# Autodesk Inventor assembly: Maquina
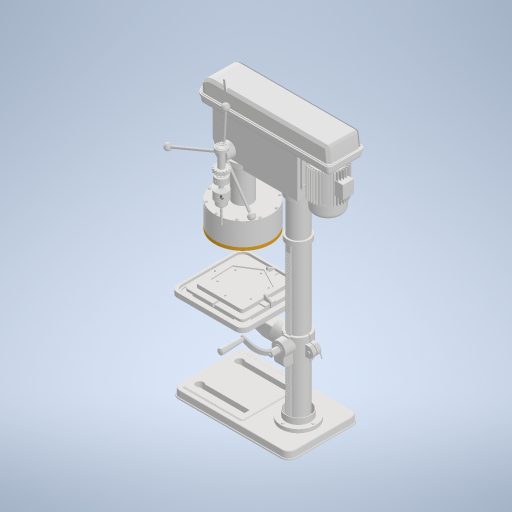
[picture p0: Inventor's stored thumbnail of the model, 512x512]
Saved by Autodesk Inventor 2024.2 (Build 282272000, 272)
## iProperties
Created: 2021-09-13
Part Number: Maquina
Description: STEP AP203
Document SubType Name: Assembly
Designer: 062210026
Sending System: SolidWorks 2018
Preprocessor: SwSTEP 2.0
Title: multi-spindle.STEP
Author: Moghimi
Revision Number: ANY
## Documents named in this file (37)
- C:\Users\062210029\Desktop\19MarV2_ProjInt3\19MarV2_ProjInt3\Maquina\Maquina.iam
- C:\Users\062210029\Desktop\19MarV2_ProjInt3\19MarV2_ProjInt3\Maquina\maquina\1_Varsay_lan.ipt
- C:\Users\062210029\Desktop\19MarV2_ProjInt3\19MarV2_ProjInt3\Maquina\maquina\2_Varsay_lan.ipt
- C:\Users\062210029\Desktop\19MarV2_ProjInt3\19MarV2_ProjInt3\Maquina\maquina\4_Varsay_lan.ipt
- C:\Users\062210029\Desktop\19MarV2_ProjInt3\19MarV2_ProjInt3\Maquina\maquina\5_Varsay_lan.ipt
- C:\Users\062210029\Desktop\19MarV2_ProjInt3\19MarV2_ProjInt3\Maquina\maquina\6_Varsay_lan.ipt
- C:\Users\062210029\Desktop\19MarV2_ProjInt3\19MarV2_ProjInt3\Maquina\maquina\7_Varsay_lan.ipt
- C:\Users\062210029\Desktop\19MarV2_ProjInt3\19MarV2_ProjInt3\Maquina\maquina\8_Varsay_lan.ipt
- C:\Users\062210029\Desktop\19MarV2_ProjInt3\19MarV2_ProjInt3\Maquina\maquina\9_Varsay_lan.ipt
- C:\Users\062210029\Desktop\19MarV2_ProjInt3\19MarV2_ProjInt3\Maquina\maquina\10_Varsay_lan.ipt
- C:\Users\062210029\Desktop\19MarV2_ProjInt3\19MarV2_ProjInt3\Maquina\maquina\11_Varsay_lan.ipt
- C:\Users\062210029\Desktop\19MarV2_ProjInt3\19MarV2_ProjInt3\Maquina\maquina\12_Varsay_lan.ipt
- C:\Users\062210029\Desktop\19MarV2_ProjInt3\19MarV2_ProjInt3\Maquina\maquina\13_Varsay_lan.ipt
- C:\Users\062210029\Desktop\19MarV2_ProjInt3\19MarV2_ProjInt3\Maquina\maquina\14_Varsay_lan.ipt
- C:\Users\062210029\Desktop\19MarV2_ProjInt3\19MarV2_ProjInt3\Maquina\maquina\15_Varsay_lan.ipt
- C:\Users\062210029\Desktop\19MarV2_ProjInt3\19MarV2_ProjInt3\Maquina\maquina\16_Varsay_lan.ipt
- C:\Users\062210029\Desktop\19MarV2_ProjInt3\19MarV2_ProjInt3\Maquina\maquina\hex bolt gradeab_iso_ISO 4014 - M4 x 35 x 14-N.ipt
- C:\Users\062210029\Desktop\19MarV2_ProjInt3\19MarV2_ProjInt3\Maquina\maquina\hex bolt gradeab_iso_ISO 4014 - M3 x 20 x 12-N.ipt
- C:\Users\062210029\Desktop\19MarV2_ProjInt3\19MarV2_ProjInt3\Maquina\maquina\hex bolt gradeab_iso_ISO 4014 - M6 x 30 x 18-N.ipt
- C:\Users\062210029\Desktop\19MarV2_ProjInt3\19MarV2_ProjInt3\Maquina\maquina\slotted cheese head screw_iso_ISO 1207 - M6 x 8 - 8N.ipt
- C:\Users\062210029\Desktop\19MarV2_ProjInt3\19MarV2_ProjInt3\Maquina\maquina\SKF_6004.iam
- C:\Users\062210029\Desktop\19MarV2_ProjInt3\19MarV2_ProjInt3\Maquina\maquina\MAILN AX.ipt
- C:\Users\062210029\Desktop\19MarV2_ProjInt3\19MarV2_ProjInt3\Maquina\maquina\SKF_30204.iam
- C:\Users\062210029\Desktop\19MarV2_ProjInt3\19MarV2_ProjInt3\Maquina\maquina\helical gear_3_am2_Metric - RH Helical gear 2.5M 30T 45HA 20PA 15FW ---30N75H50L35.0R1.ipt
- C:\Users\062210029\Desktop\19MarV2_ProjInt3\19MarV2_ProjInt3\Maquina\maquina\6-AX.ipt
- C:\Users\062210029\Desktop\19MarV2_ProjInt3\19MarV2_ProjInt3\Maquina\maquina\helical gear_3_am2_Metric - RH Helical gear 2.5M 15T 45HA 20PA 15FW ---15N75H50L25.0R1.ipt
- C:\Users\062210029\Desktop\19MarV2_ProjInt3\19MarV2_ProjInt3\Maquina\maquina\SHEL.ipt
- C:\Users\062210029\Desktop\19MarV2_ProjInt3\19MarV2_ProjInt3\Maquina\maquina\socket head cap screw_am_B18.3.1M - 5 x 0.8 x 20 Hex SHCS -- 20NHX.ipt
- C:\Users\062210029\Desktop\19MarV2_ProjInt3\19MarV2_ProjInt3\Maquina\maquina\STRIGHTER.ipt
- C:\Users\062210029\Desktop\19MarV2_ProjInt3\19MarV2_ProjInt3\Maquina\maquina\KEY.ipt
- C:\Users\062210029\Desktop\19MarV2_ProjInt3\19MarV2_ProjInt3\Maquina\maquina\spring pin slotted_ai_SPS 0.25x1.25.ipt
- C:\Users\062210029\Desktop\19MarV2_ProjInt3\19MarV2_ProjInt3\Maquina\maquina\socket head cap screw_am_B18.3.1M - 5 x 0.8 x 30 Hex SHCS -- 22NHX.ipt
- C:\Users\062210029\Desktop\19MarV2_ProjInt3\19MarV2_ProjInt3\Maquina\maquina\Drill.ipt
- C:\Users\062210029\Desktop\19MarV2_ProjInt3\19MarV2_ProjInt3\Maquina\maquina\FIXTURE.ipt
- C:\Users\062210029\Desktop\19MarV2_ProjInt3\19MarV2_ProjInt3\Maquina\maquina\WORKPICE.ipt
- C:\Users\062210029\Desktop\ProjInt3\ProjInt3\TampaBaixoFuras\TampaBaixo.ipt
- C:\Users\062210029\Desktop\Peças furadeira\Peças furadeira - Copia\Tampa_Superior.ipt
## Components (80 placed, 71 different names)
1. Tampa_Superior:1 — Mate:12, Mate:13, Mate:14, Mate:15, Mate:16, Mate:17, Mate:18, Mate:19, Mate:20, Mate:21, Mate:22, Mate:23, Mate:24, Mate:25, Mate:26, Mate:27
2. SKF_30204:7 [sub-assembly]
3. helical gear_3_am2_Metric - RH Helical gear 2.5M 15T 45HA 20PA 15FW ---15N75H50L25.0R1:7
4. 6-AX:7
5. spring pin slotted_ai_SPS 0.25x1.25:7
6. 15_Varsay_lan:8
7. Drill:7
8. 1_Varsay_lan_1
9. 2_Varsay_lan_2
10. 4_Varsay_lan_3
11. 5_Varsay_lan_4
12. 6_Varsay_lan_5
13. 7_Varsay_lan_6
14. 8_Varsay_lan_7
15. 9_Varsay_lan_8
16. 10_Varsay_lan_9
17. 11_Varsay_lan_10
18. 12_Varsay_lan_11
19. 13_Varsay_lan_12
20. 14_Varsay_lan_13
21. 14_Varsay_lan_14
22. 14_Varsay_lan_15
23. 15_Varsay_lan_16
24. 16_Varsay_lan_17
25. 16_Varsay_lan_18
26. hex bolt gradeab_iso_ISO 4014 - M4 x 35 x 14-N_19
27. hex bolt gradeab_iso_ISO 4014 - M4 x 35 x 14-N_20
28. hex bolt gradeab_iso_ISO 4014 - M4 x 35 x 14-N_21
29. hex bolt gradeab_iso_ISO 4014 - M4 x 35 x 14-N_22
30. hex bolt gradeab_iso_ISO 4014 - M3 x 20 x 12-N_23
31. hex bolt gradeab_iso_ISO 4014 - M3 x 20 x 12-N_24
32. hex bolt gradeab_iso_ISO 4014 - M3 x 20 x 12-N_25
33. hex bolt gradeab_iso_ISO 4014 - M3 x 20 x 12-N_26
34. hex bolt gradeab_iso_ISO 4014 - M6 x 30 x 18-N_27
35. hex bolt gradeab_iso_ISO 4014 - M6 x 30 x 18-N_28
36. hex bolt gradeab_iso_ISO 4014 - M6 x 30 x 18-N_29
37. hex bolt gradeab_iso_ISO 4014 - M6 x 30 x 18-N_30
38. hex bolt gradeab_iso_ISO 4014 - M6 x 30 x 18-N_31
39. slotted cheese head screw_iso_ISO 1207 - M6 x 8 - 8N_32
40. SKF_6004_34 [sub-assembly]
41. SKF_6004_35 [sub-assembly] — Mate:1
42. MAILN AX_36
43. SKF_6004_39 [sub-assembly]
44. helical gear_3_am2_Metric - RH Helical gear 2.5M 30T 45HA 20PA 15FW ---30N75H50L35.0R1_40
45. SHEL_43 — Mate:12
46. socket head cap screw_am_B18.3.1M - 5 x 0.8 x 20 Hex SHCS -- 20NHX_44 — Mate:13, Mate:14
47. STRIGHTER_46
48. KEY_47
49. SKF_6004_52 [sub-assembly]
50. SKF_6004_53 [sub-assembly]
51. socket head cap screw_am_B18.3.1M - 5 x 0.8 x 20 Hex SHCS -- 20NHX_70
52. socket head cap screw_am_B18.3.1M - 5 x 0.8 x 20 Hex SHCS -- 20NHX_71 — Mate:25, Mate:26, Mate:27
53. socket head cap screw_am_B18.3.1M - 5 x 0.8 x 20 Hex SHCS -- 20NHX_72 — Mate:23, Mate:24
54. socket head cap screw_am_B18.3.1M - 5 x 0.8 x 20 Hex SHCS -- 20NHX_73 — Mate:21, Mate:22
55. socket head cap screw_am_B18.3.1M - 5 x 0.8 x 20 Hex SHCS -- 20NHX_75 — Mate:19, Mate:20
56. socket head cap screw_am_B18.3.1M - 5 x 0.8 x 20 Hex SHCS -- 20NHX_76 — Mate:17, Mate:18
57. socket head cap screw_am_B18.3.1M - 5 x 0.8 x 20 Hex SHCS -- 20NHX_77 — Mate:15, Mate:16
58. socket head cap screw_am_B18.3.1M - 5 x 0.8 x 20 Hex SHCS -- 20NHX_78
59. socket head cap screw_am_B18.3.1M - 5 x 0.8 x 30 Hex SHCS -- 22NHX_98
60. socket head cap screw_am_B18.3.1M - 5 x 0.8 x 30 Hex SHCS -- 22NHX_99
61. socket head cap screw_am_B18.3.1M - 5 x 0.8 x 30 Hex SHCS -- 22NHX_100
62. socket head cap screw_am_B18.3.1M - 5 x 0.8 x 30 Hex SHCS -- 22NHX_101
63. socket head cap screw_am_B18.3.1M - 5 x 0.8 x 30 Hex SHCS -- 22NHX_102
64. socket head cap screw_am_B18.3.1M - 5 x 0.8 x 30 Hex SHCS -- 22NHX_103
65. socket head cap screw_am_B18.3.1M - 5 x 0.8 x 30 Hex SHCS -- 22NHX_104
66. FIXTURE_111
67. FIXTURE_112
68. WORKPICE_113
69. TampaBaixo:1 — Mate:1, Mate:3, Mate:4, Mate:5, Mate:6, Mate:7, Mate:8, Mate:9, Mate:10, Mate:11
70. socket head cap screw_am_B18.3.1M - 5 x 0.8 x 20 Hex SHCS -- 20NHX:21 — Mate:3
71. socket head cap screw_am_B18.3.1M - 5 x 0.8 x 20 Hex SHCS -- 20NHX:22 — Mate:8
72. socket head cap screw_am_B18.3.1M - 5 x 0.8 x 20 Hex SHCS -- 20NHX:23 — Mate:10
73. socket head cap screw_am_B18.3.1M - 5 x 0.8 x 20 Hex SHCS -- 20NHX:24
74. socket head cap screw_am_B18.3.1M - 5 x 0.8 x 20 Hex SHCS -- 20NHX:26 — Mate:5
75. socket head cap screw_am_B18.3.1M - 5 x 0.8 x 20 Hex SHCS -- 20NHX:27 — Mate:6
76. socket head cap screw_am_B18.3.1M - 5 x 0.8 x 20 Hex SHCS -- 20NHX:28 — Mate:9
77. socket head cap screw_am_B18.3.1M - 5 x 0.8 x 20 Hex SHCS -- 20NHX:30 — Mate:11
78. socket head cap screw_am_B18.3.1M - 5 x 0.8 x 20 Hex SHCS -- 20NHX:32 — Mate:7
79. socket head cap screw_am_B18.3.1M - 5 x 0.8 x 20 Hex SHCS -- 20NHX:33 — Mate:4
80. socket head cap screw_am_B18.3.1M - 5 x 0.8 x 20 Hex SHCS -- 20NHX_74
## Relationships (26: Mate 26)
- Mate:1: SKF_6004_35 ↔ TampaBaixo:1
- Mate:3: TampaBaixo:1 ↔ socket head cap screw_am_B18.3.1M - 5 x 0.8 x 20 Hex SHCS -- 20NHX:21
- Mate:4: TampaBaixo:1 ↔ socket head cap screw_am_B18.3.1M - 5 x 0.8 x 20 Hex SHCS -- 20NHX:33
- Mate:5: TampaBaixo:1 ↔ socket head cap screw_am_B18.3.1M - 5 x 0.8 x 20 Hex SHCS -- 20NHX:26
- Mate:6: TampaBaixo:1 ↔ socket head cap screw_am_B18.3.1M - 5 x 0.8 x 20 Hex SHCS -- 20NHX:27
- Mate:7: TampaBaixo:1 ↔ socket head cap screw_am_B18.3.1M - 5 x 0.8 x 20 Hex SHCS -- 20NHX:32
- Mate:8: TampaBaixo:1 ↔ socket head cap screw_am_B18.3.1M - 5 x 0.8 x 20 Hex SHCS -- 20NHX:22
- Mate:9: TampaBaixo:1 ↔ socket head cap screw_am_B18.3.1M - 5 x 0.8 x 20 Hex SHCS -- 20NHX:28
- Mate:10: TampaBaixo:1 ↔ socket head cap screw_am_B18.3.1M - 5 x 0.8 x 20 Hex SHCS -- 20NHX:23
- Mate:11: TampaBaixo:1 ↔ socket head cap screw_am_B18.3.1M - 5 x 0.8 x 20 Hex SHCS -- 20NHX:30
- Mate:12: Tampa_Superior:1 ↔ SHEL_43
- Mate:13: Tampa_Superior:1 ↔ socket head cap screw_am_B18.3.1M - 5 x 0.8 x 20 Hex SHCS -- 20NHX_44
- Mate:14: Tampa_Superior:1 ↔ socket head cap screw_am_B18.3.1M - 5 x 0.8 x 20 Hex SHCS -- 20NHX_44
- Mate:15: Tampa_Superior:1 ↔ socket head cap screw_am_B18.3.1M - 5 x 0.8 x 20 Hex SHCS -- 20NHX_77
- Mate:16: Tampa_Superior:1 ↔ socket head cap screw_am_B18.3.1M - 5 x 0.8 x 20 Hex SHCS -- 20NHX_77
- Mate:17: Tampa_Superior:1 ↔ socket head cap screw_am_B18.3.1M - 5 x 0.8 x 20 Hex SHCS -- 20NHX_76
- Mate:18: Tampa_Superior:1 ↔ socket head cap screw_am_B18.3.1M - 5 x 0.8 x 20 Hex SHCS -- 20NHX_76
- Mate:19: Tampa_Superior:1 ↔ socket head cap screw_am_B18.3.1M - 5 x 0.8 x 20 Hex SHCS -- 20NHX_75
- Mate:20: Tampa_Superior:1 ↔ socket head cap screw_am_B18.3.1M - 5 x 0.8 x 20 Hex SHCS -- 20NHX_75
- Mate:21: Tampa_Superior:1 ↔ socket head cap screw_am_B18.3.1M - 5 x 0.8 x 20 Hex SHCS -- 20NHX_73
- Mate:22: Tampa_Superior:1 ↔ socket head cap screw_am_B18.3.1M - 5 x 0.8 x 20 Hex SHCS -- 20NHX_73
- Mate:23: Tampa_Superior:1 ↔ socket head cap screw_am_B18.3.1M - 5 x 0.8 x 20 Hex SHCS -- 20NHX_72
- Mate:24: Tampa_Superior:1 ↔ socket head cap screw_am_B18.3.1M - 5 x 0.8 x 20 Hex SHCS -- 20NHX_72
- Mate:25: Tampa_Superior:1 ↔ socket head cap screw_am_B18.3.1M - 5 x 0.8 x 20 Hex SHCS -- 20NHX_71
- Mate:26: Tampa_Superior:1 ↔ socket head cap screw_am_B18.3.1M - 5 x 0.8 x 20 Hex SHCS -- 20NHX_71
- Mate:27: Tampa_Superior:1 ↔ socket head cap screw_am_B18.3.1M - 5 x 0.8 x 20 Hex SHCS -- 20NHX_71
